# Autodesk Inventor assembly: 00_015_FORCE_SENSOR_AMP_R1
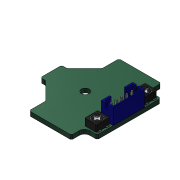
[picture p0: Inventor's stored thumbnail of the model, 180x180]
Saved by Autodesk Inventor 2021.2 (Build 252289000, 289)
## iProperties
Created: 2018-10-05
Part Number: 00_015_FORCE_SENSOR_AMP_R1
Material: 一般
Document SubType Name: Assembly
Designer: student
Mass: 1.48672 g
Surface Area: 24.0299 cm^2
Volume: 1.48672 cm^3
Density: 1 g/cm^3
Author: student
## Documents named in this file (4)
- C:\Workspace\HaptHexa\Hardware\Inventor\00_015_FORCE_SENSOR_AMP_R1.iam
- C:\Workspace\HaptHexa\Hardware\Inventor\21_017_FORCE_SENSOR_PCB_R1.ipt
- C:\Workspace\HaptHexa\Hardware\Inventor\20_016_CON_PH_5P_R1.ipt
- C:\Workspace\HaptHexa\Hardware\Inventor\20_018_SMD_VOLUME_G43A_R1.ipt
## Components (4 placed, 3 different names)
1. force_sensor_pcb:1 — メイト:1, フラッシュ:1, メイト:2, フラッシュ:2, メイト:3, フラッシュ:3
2. B5B-PH-K-S:1 — メイト:1, フラッシュ:1
3. TOCOS G43A:1 — メイト:2, フラッシュ:2
4. TOCOS G43A:2 — メイト:3, フラッシュ:3
## Relationships (6: Mate 3, Flush 3)
- メイト:1 [Mate]: force_sensor_pcb:1 ↔ B5B-PH-K-S:1
- フラッシュ:1 [Flush]: force_sensor_pcb:1 ↔ B5B-PH-K-S:1
- メイト:2 [Mate]: force_sensor_pcb:1 ↔ TOCOS G43A:1
- フラッシュ:2 [Flush] (0.5 mm): force_sensor_pcb:1 ↔ TOCOS G43A:1
- メイト:3 [Mate]: force_sensor_pcb:1 ↔ TOCOS G43A:2
- フラッシュ:3 [Flush] (0.5 mm): force_sensor_pcb:1 ↔ TOCOS G43A:2
